# Autodesk Inventor assembly: стена2
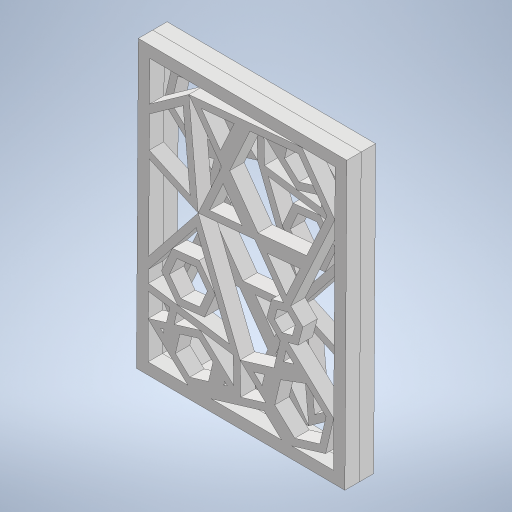
[picture p0: Inventor's stored thumbnail of the model, 512x512]
Saved by Autodesk Inventor 2023.1 (Build 271208000, 208)
## iProperties
Created: 2025-12-15
Part Number: стена2
Document SubType Name: Assembly
Designer: DELL
Author: DELL
## Documents named in this file (2)
- C:\Users\DELL\reposGitHub\VSOSH25-26\models\actuator\стена2.iam
- C:\Users\DELL\reposGitHub\VSOSH25-26\models\actuator\стена.ipt
## Components (2 placed, 1 different names)
1. стена:1 — Совмещение:1, Совмещение:2, Совмещение:3
2. стена:2 — Совмещение:1, Совмещение:2, Совмещение:3
## Relationships (3: Mate 3)
- Совмещение:1 [Mate]: стена:1 ↔ стена:2
- Совмещение:2 [Mate]: стена:1 ↔ стена:2
- Совмещение:3 [Mate]: стена:1 ↔ стена:2
